# Autodesk Inventor assembly: Frame 1647030135921
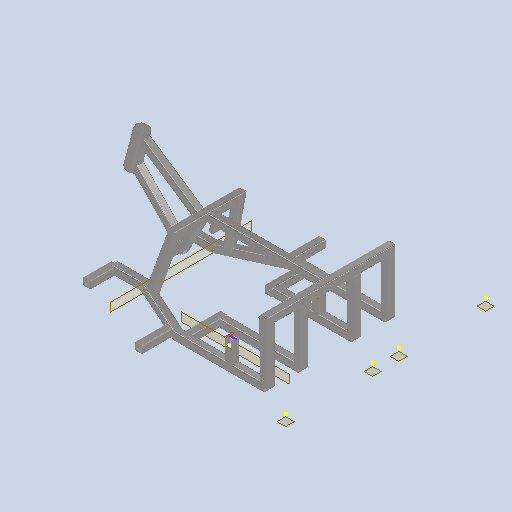
[picture p0: Inventor's stored thumbnail of the model, 512x512]
Saved by Autodesk Inventor 2022.2 (Build 262287000, 287)
## iProperties
_FrameDoc: Frame Assembly
_Version: 25.0.0
Created: 2022-03-11
Part Number: Frame 1647030135921
Document SubType Name: Assembly
Designer: foriw
Mass: 4834.2 g
Surface Area: 6123.04 cm^2
Volume: 619.192 cm^3
Density: 7.80727 g/cm^3
Author: foriw
## Documents named in this file (36)
- C:\Users\foriw\OneDrive\Dokumenter\Inventor\BeerCart - Github - Mekatronik\BeerCart-CAD-Inventor\Workspaces\Workspace\beercart assembly - mekatronik\Frame\Frame 1647030135921.iam
- C:\Users\foriw\OneDrive\Dokumenter\Inventor\BeerCart - Github - Mekatronik\BeerCart-CAD-Inventor\Workspaces\Workspace\beercart assembly - mekatronik\Frame\Skeleton 1647030135922.ipt
- C:\Users\foriw\OneDrive\Dokumenter\Inventor\BeerCart - Github - Mekatronik\BeerCart-CAD-Inventor\Workspaces\Workspace\beercart assembly - mekatronik\Frame\ISO 12633-2 20x20x2 1647030137505.ipt
- C:\Users\foriw\OneDrive\Dokumenter\Inventor\BeerCart - Github - Mekatronik\BeerCart-CAD-Inventor\Workspaces\Workspace\beercart assembly - mekatronik\Frame\ISO 12633-2 20x20x2 1647030137863.ipt
- C:\Users\foriw\OneDrive\Dokumenter\Inventor\BeerCart - Github - Mekatronik\BeerCart-CAD-Inventor\Workspaces\Workspace\beercart assembly - mekatronik\Frame\ISO 12633-2 20x20x2 1647030137981.ipt
- C:\Users\foriw\OneDrive\Dokumenter\Inventor\BeerCart - Github - Mekatronik\BeerCart-CAD-Inventor\Workspaces\Workspace\beercart assembly - mekatronik\Frame\ISO 12633-2 20x20x2 1647030138110.ipt
- C:\Users\foriw\OneDrive\Dokumenter\Inventor\BeerCart - Github - Mekatronik\BeerCart-CAD-Inventor\Workspaces\Workspace\beercart assembly - mekatronik\Frame\ISO 12633-2 20x20x2 1647030138225.ipt
- C:\Users\foriw\OneDrive\Dokumenter\Inventor\BeerCart - Github - Mekatronik\BeerCart-CAD-Inventor\Workspaces\Workspace\beercart assembly - mekatronik\Frame\ISO 12633-2 20x20x2 1647030639616.ipt
- C:\Users\foriw\OneDrive\Dokumenter\Inventor\BeerCart - Github - Mekatronik\BeerCart-CAD-Inventor\Workspaces\Workspace\beercart assembly - mekatronik\Frame\ISO 12633-2 20x20x2 1647030639707.ipt
- C:\Users\foriw\OneDrive\Dokumenter\Inventor\BeerCart - Github - Mekatronik\BeerCart-CAD-Inventor\Workspaces\Workspace\beercart assembly - mekatronik\Frame\ISO 1035_2 10x 10 1647602096505.ipt
- C:\Users\foriw\OneDrive\Dokumenter\Inventor\BeerCart - Github - Mekatronik\BeerCart-CAD-Inventor\Workspaces\Workspace\beercart assembly - mekatronik\Frame\ISO 1035_2 10x 10 1647602096566.ipt
- C:\Users\foriw\OneDrive\Dokumenter\Inventor\BeerCart - Github - Mekatronik\BeerCart-CAD-Inventor\Workspaces\Workspace\beercart assembly - mekatronik\Frame\ISO 1035_2 10x 10 1647602096620.ipt
- C:\Users\foriw\OneDrive\Dokumenter\Inventor\BeerCart - Github - Mekatronik\BeerCart-CAD-Inventor\Workspaces\Workspace\beercart assembly - mekatronik\Frame\ISO 12633-2 20x20x2 1647606064149.ipt
- C:\Users\foriw\OneDrive\Dokumenter\Inventor\BeerCart - Github - Mekatronik\BeerCart-CAD-Inventor\Workspaces\Workspace\beercart assembly - mekatronik\Frame\ISO 12633-2 20x20x2 1647606064205.ipt
- C:\Users\foriw\OneDrive\Dokumenter\Inventor\BeerCart - Github - Mekatronik\BeerCart-CAD-Inventor\Workspaces\Workspace\beercart assembly - mekatronik\Frame\ISO 12633-2 20x20x2 1647606177319.ipt
- C:\Users\foriw\OneDrive\Dokumenter\Inventor\BeerCart - Github - Mekatronik\BeerCart-CAD-Inventor\Workspaces\Workspace\beercart assembly - mekatronik\Frame\ISO 12633-2 20x20x2 1647606177438.ipt
- C:\Users\foriw\OneDrive\Dokumenter\Inventor\BeerCart - Github - Mekatronik\BeerCart-CAD-Inventor\Workspaces\Workspace\beercart assembly - mekatronik\Frame\ISO 12633-2 20x20x2 1648114433069.ipt
- C:\Users\foriw\OneDrive\Dokumenter\Inventor\BeerCart - Github - Mekatronik\BeerCart-CAD-Inventor\Workspaces\Workspace\beercart assembly - mekatronik\Frame\ISO 12633-2 20x20x2 1648114433206.ipt
- C:\Users\foriw\OneDrive\Dokumenter\Inventor\BeerCart - Github - Mekatronik\BeerCart-CAD-Inventor\Workspaces\Workspace\beercart assembly - mekatronik\Frame\FrontWheelFrame.iam
- C:\Users\foriw\OneDrive\Dokumenter\Inventor\BeerCart - Github - Mekatronik\BeerCart-CAD-Inventor\Workspaces\Workspace\beercart assembly - mekatronik\Frame\ISO 12633-2 20x20x2 1648198059381.ipt
- C:\Users\foriw\OneDrive\Dokumenter\Inventor\BeerCart - Github - Mekatronik\BeerCart-CAD-Inventor\Workspaces\Workspace\beercart assembly - mekatronik\Frame\ISO 12633-2 20x20x2 1648210122818.ipt
- C:\Users\foriw\OneDrive\Dokumenter\Inventor\BeerCart - Github - Mekatronik\BeerCart-CAD-Inventor\Workspaces\Workspace\beercart assembly - mekatronik\Frame\ISO 12633-2 20x20x2 1648210122933.ipt
- C:\Users\foriw\OneDrive\Dokumenter\Inventor\BeerCart - Github - Mekatronik\BeerCart-CAD-Inventor\Workspaces\Workspace\beercart assembly - mekatronik\Frame\ISO 12633-2 20x20x2 1648210123049.ipt
- C:\Users\foriw\OneDrive\Dokumenter\Inventor\BeerCart - Github - Mekatronik\BeerCart-CAD-Inventor\Workspaces\Workspace\beercart assembly - mekatronik\Frame\ISO 12633-2 20x20x2 1648210123162.ipt
- C:\Users\foriw\OneDrive\Dokumenter\Inventor\BeerCart - Github - Mekatronik\BeerCart-CAD-Inventor\Workspaces\Workspace\BackWheelMountingPlate.ipt
- C:\Users\foriw\OneDrive\Dokumenter\Inventor\BeerCart - Github - Mekatronik\BeerCart-CAD-Inventor\Workspaces\Workspace\BackWheelMountingPlate_MIR.ipt
- C:\Users\foriw\OneDrive\Dokumenter\Inventor\BeerCart - Github - Mekatronik\BeerCart-CAD-Inventor\Workspaces\Workspace\BackWheelMountingPlate_MIR1.ipt
- C:\Users\foriw\OneDrive\Dokumenter\Inventor\BeerCart - Github - Mekatronik\BeerCart-CAD-Inventor\Workspaces\Workspace\BackWheelMountingPlate_MIR_MIR.ipt
- C:\Users\foriw\OneDrive\Dokumenter\Inventor\BeerCart - Github - Mekatronik\BeerCart-CAD-Inventor\Workspaces\Workspace\beercart assembly - mekatronik\Frame\ISO 1035_2 10x 10 1648211737860.ipt
- C:\Users\foriw\OneDrive\Dokumenter\Inventor\BeerCart - Github - Mekatronik\BeerCart-CAD-Inventor\Workspaces\Workspace\bearing housing front.ipt
- C:\Users\foriw\OneDrive\Dokumenter\Inventor\BeerCart - Github - Mekatronik\BeerCart-CAD-Inventor\Workspaces\Workspace\beercart assembly - mekatronik\Frame\ISO 12633-2 20x20x2 1648404911470.ipt
- C:\Users\foriw\OneDrive\Dokumenter\Inventor\BeerCart - Github - Mekatronik\BeerCart-CAD-Inventor\Workspaces\Workspace\beercart assembly - mekatronik\Frame\ISO 12633-2 20x20x2 1648404911558.ipt
- C:\Users\foriw\OneDrive\Dokumenter\Inventor\BeerCart - Github - Mekatronik\BeerCart-CAD-Inventor\Workspaces\Workspace\beercart assembly - mekatronik\Frame\ISO 12633-2 20x20x2 1648404911659.ipt
- C:\Users\foriw\OneDrive\Dokumenter\Inventor\BeerCart - Github - Mekatronik\BeerCart-CAD-Inventor\Workspaces\Workspace\beercart assembly - mekatronik\Frame\ISO 12633-2 20x20x2 1648404911754.ipt
- C:\Users\foriw\OneDrive\Dokumenter\Inventor\BeerCart - Github - Mekatronik\BeerCart-CAD-Inventor\Workspaces\Workspace\beercart assembly - mekatronik\Frame\ISO 12633-2 20x20x2 1648404911848.ipt
- C:\Users\foriw\OneDrive\Dokumenter\Inventor\BeerCart - Github - Mekatronik\BeerCart-CAD-Inventor\Workspaces\Workspace\beercart assembly - mekatronik\Frame\ISO 12633-2 20x20x2 1648404911940.ipt
## Components (38 placed, 22 different names)
1. bearing housing front:1 — Rotational:1
2. Reference Skeleton
3. ISO 12633-2 20x20x2 - 329.48:2
4. ISO 12633-2 20x20x2 - 159,65:1
5. ISO 12633-2 20x20x2 - 159,65:2
6. ISO 12633-2 20x20x2 - 290:1
7. ISO 12633-2 20x20x2 - 185.38:3
8. ISO 12633-2 20x20x2 - 166.84:1
9. ISO 12633-2 20x20x2 - 166.84:2
10. ISO 1035/2 10x 10 - 58.59:1
11. ISO 1035/2 10x 10 - 43.59:1
12. ISO 1035/2 10x 10 - 43.59:2
13. ISO 12633-2 20x20x2 - 231.89:1
14. ISO 12633-2 20x20x2 - 231.89:2 — Symmetry:1
15. ISO 12633-2 20x20x2 - 166.38:1 — Mate:1, Mate:3
16. ISO 12633-2 20x20x2 - 166.38:2 — Mate:2, Mate:4, Mate:5
17. ISO 12633-2 20x20x2 - 140:1
18. ISO 12633-2 20x20x2 - 140:2
19. BackWheelMountingPlate:1
20. FrontWheelFrame:1 [sub-assembly] — Rotational:1
21. ISO 12633-2 20x20x2 - 54:1
22. ISO 12633-2 20x20x2 - 200:1 — Symmetry:1
23. ISO 12633-2 20x20x2 - 97:1
24. ISO 12633-2 20x20x2 - 200:2
25. ISO 12633-2 20x20x2 - 97:2
26. BackWheelMountingPlate_MIR:1 — Mate:7, Mate:8, Mate:9
27. ISO 12633-2 20x20x2 - 54:2 — Mate:7, Mate:8, Mate:9
28. BackWheelMountingPlate_MIR1:1 — Mate:10, Mate:11, Mate:12
29. ISO 12633-2 20x20x2 - 54:3 — Mate:10, Mate:11, Mate:12
30. BackWheelMountingPlate_MIR_MIR:1 — Mate:13, Flush:3, Flush:4
31. ISO 12633-2 20x20x2 - 54:4 — Mate:13, Flush:3, Flush:4
32. ISO 1035/2 10x 10 - 58.59:1
33. ISO 12633-2 20x20x2 - 80:1
34. ISO 12633-2 20x20x2 - 80:2
35. ISO 12633-2 20x20x2 - 80:3
36. ISO 12633-2 20x20x2 - 70:1
37. ISO 12633-2 20x20x2 - 80:4
38. ISO 12633-2 20x20x2 - 70:2
## Relationships (21: Mate 14, Flush 5, Symmetry 1, RevoluteJoint 1)
- Mate:1: ISO 12633-2 20x20x2 - 166.38:1
- Mate:2: ISO 12633-2 20x20x2 - 166.38:2
- Mate:3: ISO 12633-2 20x20x2 - 166.38:1
- Mate:4: ISO 12633-2 20x20x2 - 166.38:2
- Mate:5: ISO 12633-2 20x20x2 - 166.38:2
- Symmetry:1: ISO 12633-2 20x20x2 - 231.89:2 ↔ ISO 12633-2 20x20x2 - 200:1
- [Mate]: BackWheelMountingPlate:1 ↔ ISO 12633-2 20x20x2 - 54:1
- [Flush]: BackWheelMountingPlate:1 ↔ ISO 12633-2 20x20x2 - 54:1
- [Flush]: BackWheelMountingPlate:1 ↔ ISO 12633-2 20x20x2 - 54:1
- Mate:7: BackWheelMountingPlate_MIR:1 ↔ ISO 12633-2 20x20x2 - 54:2
- Mate:8: BackWheelMountingPlate_MIR:1 ↔ ISO 12633-2 20x20x2 - 54:2
- Mate:9: BackWheelMountingPlate_MIR:1 ↔ ISO 12633-2 20x20x2 - 54:2
- Mate:10: BackWheelMountingPlate_MIR1:1 ↔ ISO 12633-2 20x20x2 - 54:3
- Mate:11: BackWheelMountingPlate_MIR1:1 ↔ ISO 12633-2 20x20x2 - 54:3
- Mate:12: BackWheelMountingPlate_MIR1:1 ↔ ISO 12633-2 20x20x2 - 54:3
- Mate:13: BackWheelMountingPlate_MIR_MIR:1 ↔ ISO 12633-2 20x20x2 - 54:4
- Flush:3: BackWheelMountingPlate_MIR_MIR:1 ↔ ISO 12633-2 20x20x2 - 54:4
- Flush:4: BackWheelMountingPlate_MIR_MIR:1 ↔ ISO 12633-2 20x20x2 - 54:4
- [Mate]: bearing housing front:1 ↔ ISO 1035/2 10x 10 - 58.59:1
- [Flush] (1 mm): bearing housing front:1 ↔ ISO 1035/2 10x 10 - 58.59:1
- Rotational:1 [RevoluteJoint] (4 mm): bearing housing front:1 ↔ FrontWheelFrame:1
## Named parameters: d22_d2 = 0 mm, d23_d3 = 1 mm
